# Autodesk Inventor assembly: centre wing
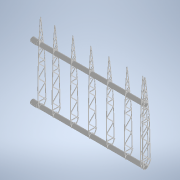
[picture p0: Inventor's stored thumbnail of the model, 180x180]
Saved by Autodesk Inventor 2022 (Build 260153000, 153)
## iProperties
Created: 2021-03-09
Part Number: centre wing
Document SubType Name: Assembly
Designer: Ferdinand Hubbard
Author: Ferdinand Hubbard
## Documents named in this file (4)
- C:\Users\Ferdinand Hubbard\Desktop\solarplane\cad\left wing section.iam
- C:\Users\Ferdinand Hubbard\Desktop\solarplane\cad\tubes\normal tubes\18mm tube.ipt
- C:\Users\Ferdinand Hubbard\Desktop\solarplane\cad\airfoils\full airfoil\full airfoil blueprint 19 mm.ipt
- C:\Users\Ferdinand Hubbard\Desktop\solarplane\cad\tubes\normal tubes\angle connector 19 mm.ipt
## Components (12 placed, 3 different names)
1. 18mm tube:1 — Angle:2, Mate:10, Flush:2, Mate:25, Mate:26
2. 18mm tube:2 — Angle:1, Mate:11, Flush:1, Flush:3, Mate:23, Mate:24
3. full airfoil blueprint 19 mm:2 — Mate:1, Mate:2, Mate:3, Angle:1, Angle:2, Mate:10, Mate:11, Flush:1, Flush:2, Mate:21, Mate:22
4. full airfoil blueprint 19 mm:3 — Mate:1, Mate:2, Mate:3, Mate:7, Mate:8, Mate:9
5. full airfoil blueprint 19 mm:4 — Mate:7, Mate:8, Mate:9
6. full airfoil blueprint 19 mm:5 — Mate:18, Mate:19, Mate:20
7. full airfoil blueprint 19 mm:6 — Mate:18, Mate:19, Mate:20
8. full airfoil blueprint 19 mm:7
9. full airfoil blueprint 19 mm:8
10. full airfoil blueprint 19 mm:9 — Flush:3, Mate:21, Mate:22
11. angle connector 19 mm:1 — Mate:23, Mate:24
12. angle connector 19 mm:2 — Mate:25, Mate:26
## Relationships (30: Mate 25, Flush 3, Angle 2)
- Mate:1 (80 mm): full airfoil blueprint 19 mm:2 ↔ full airfoil blueprint 19 mm:3
- Mate:2: full airfoil blueprint 19 mm:2 ↔ full airfoil blueprint 19 mm:3
- Mate:3: full airfoil blueprint 19 mm:2 ↔ full airfoil blueprint 19 mm:3
- [Mate] (80 mm): full airfoil blueprint 19 mm:4 ↔ full airfoil blueprint 19 mm:5
- [Mate]: full airfoil blueprint 19 mm:4 ↔ full airfoil blueprint 19 mm:5
- [Mate]: full airfoil blueprint 19 mm:4 ↔ full airfoil blueprint 19 mm:5
- Mate:7: full airfoil blueprint 19 mm:3 ↔ full airfoil blueprint 19 mm:4
- Mate:8: full airfoil blueprint 19 mm:3 ↔ full airfoil blueprint 19 mm:4
- Mate:9 (80 mm): full airfoil blueprint 19 mm:3 ↔ full airfoil blueprint 19 mm:4
- Angle:1 (180 deg): 18mm tube:2 ↔ full airfoil blueprint 19 mm:2
- Angle:2 (180 deg): 18mm tube:1 ↔ full airfoil blueprint 19 mm:2
- Mate:10: 18mm tube:1 ↔ full airfoil blueprint 19 mm:2
- Mate:11: 18mm tube:2 ↔ full airfoil blueprint 19 mm:2
- Flush:1: 18mm tube:2 ↔ full airfoil blueprint 19 mm:2
- Flush:2: 18mm tube:1 ↔ full airfoil blueprint 19 mm:2
- [Mate]: full airfoil blueprint 19 mm:7 ↔ full airfoil blueprint 19 mm:8
- [Mate]: full airfoil blueprint 19 mm:7 ↔ full airfoil blueprint 19 mm:8
- [Mate]: full airfoil blueprint 19 mm:6 ↔ full airfoil blueprint 19 mm:7
- [Mate]: full airfoil blueprint 19 mm:6 ↔ full airfoil blueprint 19 mm:7
- [Mate] (80 mm): full airfoil blueprint 19 mm:6 ↔ full airfoil blueprint 19 mm:7
- Mate:18 (80 mm): full airfoil blueprint 19 mm:5 ↔ full airfoil blueprint 19 mm:6
- Mate:19: full airfoil blueprint 19 mm:5 ↔ full airfoil blueprint 19 mm:6
- Mate:20: full airfoil blueprint 19 mm:5 ↔ full airfoil blueprint 19 mm:6
- Flush:3 (10 mm): 18mm tube:2 ↔ full airfoil blueprint 19 mm:9
- Mate:21: full airfoil blueprint 19 mm:2 ↔ full airfoil blueprint 19 mm:9
- Mate:22: full airfoil blueprint 19 mm:2 ↔ full airfoil blueprint 19 mm:9
- Mate:23: 18mm tube:2 ↔ angle connector 19 mm:1
- Mate:24: 18mm tube:2 ↔ angle connector 19 mm:1
- Mate:25: 18mm tube:1 ↔ angle connector 19 mm:2
- Mate:26: 18mm tube:1 ↔ angle connector 19 mm:2
## Named parameters: d440_d437 = 80 mm, d441_d438 = 0 mm, d442_d439 = 0 mm, d453_d441_d438 = 0 mm, d454_d442_d439 = 0 mm, d455_d443 = 0 mm, d456_d444 = 0 mm, d457_d445 = 80 mm
